# Autodesk Inventor assembly: CLB_077_ScissorTopBarAssembly
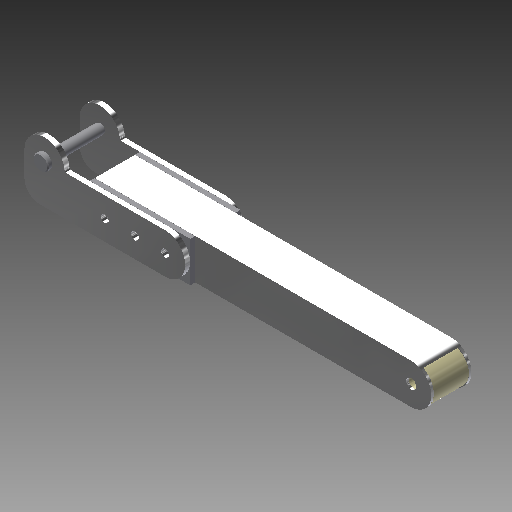
[picture p0: Inventor's stored thumbnail of the model, 512x512]
Saved by Autodesk Inventor 2018 (Build 220112000, 112)
## iProperties
Created: 2020-02-13
Part Number: CLB_077_ScissorTopBarAssembly
Document SubType Name: Assembly
Designer: Cooper
Author: Cooper
## Documents named in this file (8)
- C:\Users\Cooper\Documents\GrabCAD\Infinite Recharge 2020\Build season\CLB_077_ScissorTopBarAssembly.iam
- C:\Users\Cooper\Documents\GrabCAD\Infinite Recharge 2020\Build season\CLB_036_FourPartScissorBarTop.ipt
- C:\Users\Cooper\Documents\GrabCAD\Infinite Recharge 2020\Build season\CLB_027_LifterBracket.ipt
- C:\Users\Cooper\Documents\GrabCAD\Infinite Recharge 2020\Build season\CLB_053_ScissorTopBarPlug.ipt
- C:\Users\Cooper\Documents\GrabCAD\Infinite Recharge 2020\Build season\CLB_052_ScissorLiftPlug.ipt
- C:\Users\Cooper\Documents\GrabCAD\Infinite Recharge 2020\Build season\CLB_040_ScissorLiftSpacer2.ipt
- C:\Users\Cooper\Documents\GrabCAD\Infinite Recharge 2020\Build season\CLB_046_ClevisPinScissors.ipt
- CLB_027_LifterBracket.ipt
## Components (8 placed, 6 different names)
1. CLB_036_FourPartScissorBarTop:1 — Flush:37, Flush:38, Flush:39, Mate:31, Mate:32, Flush:44, Mate:33, Flush:45, Mate:34, Mate:35, Mate:36, Flush:47, Mate:37, Mate:38
2. CLB_027_LifterBracket:9 — Flush:38, Flush:46, Flush:48, Insert:4
3. CLB_027_LifterBracket:10 — Flush:37, Flush:39, Flush:46, Insert:2, Insert:5
4. CLB_053_ScissorTopBarPlug:1 — Mate:31, Mate:32, Flush:44
5. CLB_052_ScissorLiftPlug:2 — Mate:33, Flush:45, Mate:34, Mate:35
6. CLB_040_ScissorLiftSpacer2:1 — Flush:47, Insert:2, Mate:37
7. CLB_040_ScissorLiftSpacer2:2 — Flush:48, Insert:4, Mate:38
8. CLB_046_ClevisPinScissors:1 — Insert:5
## Relationships (19: Flush 8, Mate 8, Insert 3)
- Flush:37: CLB_036_FourPartScissorBarTop:1 ↔ CLB_027_LifterBracket:10
- Flush:38: CLB_036_FourPartScissorBarTop:1 ↔ CLB_027_LifterBracket:9
- Flush:39 (-38.1 mm): CLB_036_FourPartScissorBarTop:1 ↔ CLB_027_LifterBracket:10
- Mate:31: CLB_036_FourPartScissorBarTop:1 ↔ CLB_053_ScissorTopBarPlug:1
- Mate:32: CLB_036_FourPartScissorBarTop:1 ↔ CLB_053_ScissorTopBarPlug:1
- Flush:44 (176.2125 mm): CLB_036_FourPartScissorBarTop:1 ↔ CLB_053_ScissorTopBarPlug:1
- Mate:33: CLB_036_FourPartScissorBarTop:1 ↔ CLB_052_ScissorLiftPlug:2
- Flush:45: CLB_036_FourPartScissorBarTop:1 ↔ CLB_052_ScissorLiftPlug:2
- Mate:34: CLB_036_FourPartScissorBarTop:1 ↔ CLB_052_ScissorLiftPlug:2
- Mate:35: CLB_036_FourPartScissorBarTop:1 ↔ CLB_052_ScissorLiftPlug:2
- Mate:36: CLB_036_FourPartScissorBarTop:1
- Flush:46: CLB_027_LifterBracket:9 ↔ CLB_027_LifterBracket:10
- Flush:47: CLB_036_FourPartScissorBarTop:1 ↔ CLB_040_ScissorLiftSpacer2:1
- Insert:2: CLB_027_LifterBracket:10 ↔ CLB_040_ScissorLiftSpacer2:1
- Flush:48: CLB_027_LifterBracket:9 ↔ CLB_040_ScissorLiftSpacer2:2
- Insert:4: CLB_027_LifterBracket:9 ↔ CLB_040_ScissorLiftSpacer2:2
- Mate:37: CLB_036_FourPartScissorBarTop:1 ↔ CLB_040_ScissorLiftSpacer2:1
- Mate:38: CLB_036_FourPartScissorBarTop:1 ↔ CLB_040_ScissorLiftSpacer2:2
- Insert:5: CLB_027_LifterBracket:10 ↔ CLB_046_ClevisPinScissors:1
